# Autodesk Inventor assembly: Chuck Assembly
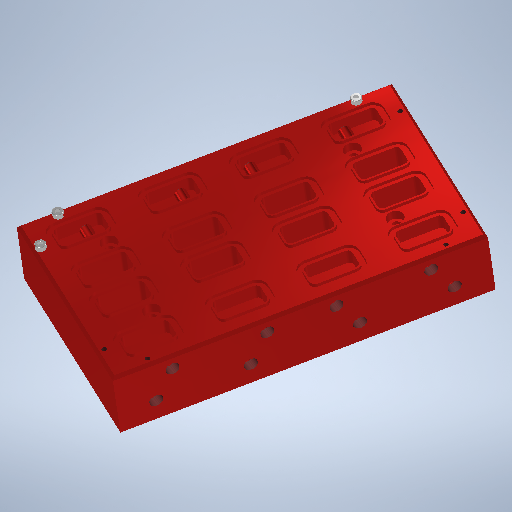
[picture p0: Inventor's stored thumbnail of the model, 512x512]
Saved by Autodesk Inventor 2025 (Build 290162000, 162)
## iProperties
Created: 2021-01-11
Part Number: Chuck Assembly
Document SubType Name: Assembly
Designer: caleb
Author: caleb
## Documents named in this file (3)
- C:\Users\cfang\Desktop\nebraska-silicon-lab\Hardware\ETL\Module Assembly\Chuck - 16-pocket V1\Chuck - 16-pocket.iam
- C:\Users\cfang\Desktop\nebraska-silicon-lab\Hardware\ETL\Module Assembly\Chuck - 16-pocket V1\90128A212_ZNC-PLTD ALLOY STL SCKT HEAD CAP SCREW.ipt
- C:\Users\cfang\Desktop\nebraska-silicon-lab\Hardware\ETL\Module Assembly\Chuck - 16-pocket V1\Chuck - 16-pocket.ipt
## Components (4 placed, 2 different names)
1. Chuck - 16-pocket:1 — Insert:1, Insert:2, Insert:3
2. 90128A212_ZNC-PLTD ALLOY STL SCKT HEAD CAP SCREW:1 — Insert:2
3. 90128A212_ZNC-PLTD ALLOY STL SCKT HEAD CAP SCREW:2 — Insert:3
4. 90128A212_ZNC-PLTD ALLOY STL SCKT HEAD CAP SCREW:3 — Insert:1
## Relationships (3: Insert 3)
- Insert:1: Chuck - 16-pocket:1 ↔ 90128A212_ZNC-PLTD ALLOY STL SCKT HEAD CAP SCREW:3
- Insert:2: Chuck - 16-pocket:1 ↔ 90128A212_ZNC-PLTD ALLOY STL SCKT HEAD CAP SCREW:1
- Insert:3: Chuck - 16-pocket:1 ↔ 90128A212_ZNC-PLTD ALLOY STL SCKT HEAD CAP SCREW:2
